# Autodesk Inventor assembly: SSCSW10-8
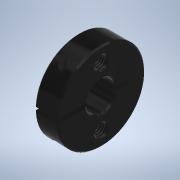
[picture p0: Inventor's stored thumbnail of the model, 180x180]
Saved by Autodesk Inventor 2021 (Build 250183000, 183)
## iProperties
Category: PARTsolutions
Company: MISUMI
Part Number: SSCSW10-8
Catalog Web Link: www.cadenas.de
Description: SCSW, PSCSW, SSCSW-Shaft Collars - 2-Tapped (Coarse Thread)
Vendor: MISUMI
Document SubType Name: Assembly
Designer: partserver
Manufacturer: MISUMI
Mass: 4.45258 g
Surface Area: 29.1469 cm^2
Volume: 4.45258 cm^3
Density: 1 g/cm^3
PSOL_IDENT_0: {$CADENAS_DATA\23d-libs\misumi\metric\03_set_collars\scsw_asmtab.prj},195 {VTYP=3D},{STYP=ASSTAB},{N
PSOL_IDENT_1: B=SSCSW10-8},{LINA=SSCSW10-8},{NN=SCSW, PSCSW, SSCSW},{DATE=09.09.2019 15:26:50},{GEOMDATE=24.02.201
PSOL_IDENT_2: 6 04:35:42},{VERSION=},{LINEID=60},{WBVAR=MAT,ST,BS},{WBNUMERIC=BS}  {NB=SSCSW10-8},{LINA=SSCSW10-8}
PSOL_IDENT_3: ,{KT=DUMMY},{PN=SSCSW10-8},{TYPE=SSCSW},{MAT=304},{ST=-},{AC=Hexagon Socket Head Set Screw 1 Pc. (30
PSOL_IDENT_4: 4 Stainless Steel) },{D=10},{BS=8},{D1=30},{M=M3},{THMD=3},{THDMIN=2.459},{ST0='-','-'},{B1=8,10,12}
PSOL_IDENT_5: ,{DD=3.4},{R=3.00},{W=1.5},{X=9.0},{Y=5.0},{Z=8~10},{S=5.5},{P=20},{C=0.5},{L=10},{M1=M5},{ZZ=9},{TH
PSOL_IDENT_6: MD1=5},{THDMIN1=4.134},{PPATH=scsw_templ.prj}
NB: SSCSW10-8
NN: SCSW, PSCSW, SSCSW
NT: Shaft Collars - 2-Tapped (Coarse Thread)
NBSYN: $PN.
LINA: SSCSW10-8
CATALOG: Misumi
PN: SSCSW10-8
MAT: SUS304 Equivalent
ST: -
AC: Hexagon Socket Head Set Screw 1 Pc. (304 Stainless Steel)
D: 10
BS: 8
D1: 30
M: M3
DD: 3.4
R: 3
W: 1.5
X: 9
Y: 5
Z: 8~10
S: 5.5
P: 20
M1: M5
SUPPLIER: MISUMI
ARTICLENO: SSCSW10-8
BOMINFO: SSCSW10-8
CREATOR: CADENAS GmbH
Title: SSCSW10-8
Author: Cadenas PARTsolutions
Comments: Shaft Collars - 2-Tapped (Coarse Thread)
## Documents named in this file (3)
- C:\Users\Hagihara Yuya\Documents\Inventor\Projects\NHK2021\DoRa-Chan\SetColor\SSCSW10-8\SSCSW10-8.iam
- C:\Users\Hagihara Yuya\Documents\Inventor\Projects\NHK2021\DoRa-Chan\SetColor\SSCSW10-8\SSCSW10-8b.ipt
- C:\Users\Hagihara Yuya\Documents\Inventor\Projects\NHK2021\DoRa-Chan\SetColor\SSCSW10-8\Slotted head cap screw ISO 4762 - M3x10.ipt
## Components (2 placed, 2 different names)
1. SSCSW10-8b:1 — body_screw_Z@1 <-> IP1_Z@2
2. Slotted head cap screw ISO 4762 - M3x10:1 — body_screw_Z@1 <-> IP1_Z@2
## Relationships (1: Mate 1)
- body_screw_Z@1 <-> IP1_Z@2 [Mate]: SSCSW10-8b:1 ↔ Slotted head cap screw ISO 4762 - M3x10:1
